# Autodesk Inventor assembly: Projekat
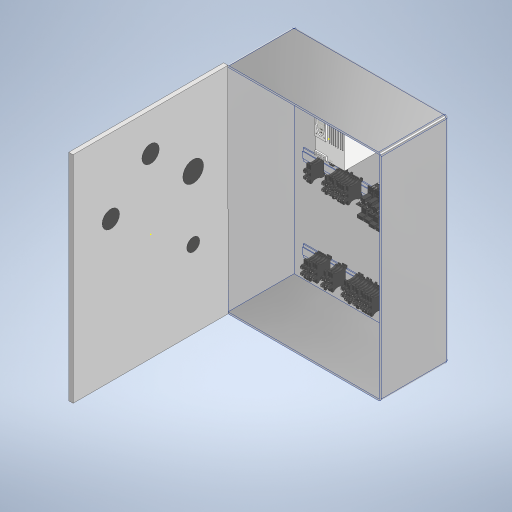
[picture p0: Inventor's stored thumbnail of the model, 512x512]
Saved by Autodesk Inventor 2023 (Build 270158000, 158)
## iProperties
Created: 2022-07-07
Part Number: Projekat
Document SubType Name: Assembly
Designer: User
Author: User
## Documents named in this file (9)
- C:\Users\User\Desktop\PMS\Seminarski rad\Inventor_sheme\Projekat.iam
- C:\Users\User\Desktop\PMS\Seminarski rad\Inventor_sheme\Ormar.ipt
- C:\Users\User\Desktop\PMS\Seminarski rad\Inventor_sheme\vrata.ipt
- C:\Users\User\Desktop\PMS\Seminarski rad\manja_sklopka\a9f89116.iam
- C:\Users\User\Desktop\PMS\Seminarski rad\Inventor_sheme\redna_stezaljka.ipt
- C:\Users\User\Desktop\PMS\Seminarski rad\sklopka\domf01204.iam
- C:\Users\User\Desktop\PMS\Seminarski rad\Inventor_sheme\napojna_jedinica_ABL8RPS24100.ipt
- C:\Users\User\Desktop\PMS\Seminarski rad\odvodnik_prenapona\a9a26500.iam
- C:\Users\User\Desktop\PMS\Seminarski rad\rsb_relay\rsb1a120f7pv.ipt
## Components (63 placed, 8 different names)
1. Ormar:1 — Mate:1, Mate:4, Mate:5, Mate:7, Mate:8, Mate:9, Mate:10, Mate:11, Mate:12, Mate:13, Mate:14, Mate:15, Mate:16, Mate:17, Mate:18, Mate:19, Mate:20, Mate:21, Mate:22, Mate:23, Mate:24, Mate:25, Mate:26, Mate:27, Mate:28, Mate:29, Mate:30, Mate:31, Mate:32, Mate:33, Mate:34, Mate:35, Mate:36, Mate:37, Mate:38, Mate:39, Mate:40, Mate:41, Mate:42, Mate:43, Mate:44, Mate:45, Mate:46, Mate:47, Mate:48, Mate:49, Mate:50, Mate:51, Mate:52, Mate:53, Mate:54, Mate:55, Mate:56, Mate:57, Mate:58, Mate:59, Mate:60, Mate:61, Mate:62, Mate:63, Mate:64, Mate:65, Mate:66
2. a9a26500:1 [sub-assembly] — Mate:8
3. domf01204:1 [sub-assembly] — Mate:5
4. a9f89116:1 [sub-assembly] — Mate:7
5. napojna_jedinica_ABL8RPS24100:1 — Mate:4
6. vrata:1 — Mate:1
7. redna_stezaljka:1 — Mate:9, Mate:11
8. redna_stezaljka:2 — Mate:10
9. redna_stezaljka:3 — Mate:12
10. redna_stezaljka:4 — Mate:13
11. redna_stezaljka:5 — Mate:15
12. redna_stezaljka:6 — Mate:16
13. redna_stezaljka:7 — Mate:14
14. redna_stezaljka:8 — Mate:24
15. redna_stezaljka:9 — Mate:23
16. redna_stezaljka:10 — Mate:21
17. redna_stezaljka:11 — Mate:22
18. redna_stezaljka:12 — Mate:17
19. redna_stezaljka:13 — Mate:20
20. redna_stezaljka:14 — Mate:18
21. redna_stezaljka:15 — Mate:19
22. rsb1a120f7pv:1 — Mate:25
23. rsb1a120f7pv:4 — Mate:26
24. rsb1a120f7pv:5 — Mate:27
25. rsb1a120f7pv:6 — Mate:28
26. rsb1a120f7pv:7 — Mate:29
27. rsb1a120f7pv:8 — Mate:30
28. redna_stezaljka:16 — Mate:39
29. redna_stezaljka:17 — Mate:36
30. redna_stezaljka:18 — Mate:35
31. redna_stezaljka:19 — Mate:38
32. redna_stezaljka:20 — Mate:40
33. redna_stezaljka:21 — Mate:41
34. redna_stezaljka:22 — Mate:37
35. redna_stezaljka:23 — Mate:34
36. redna_stezaljka:24 — Mate:33
37. redna_stezaljka:25 — Mate:31
38. redna_stezaljka:26 — Mate:32
39. redna_stezaljka:27 — Mate:47
40. redna_stezaljka:28 — Mate:48
41. redna_stezaljka:29 — Mate:46
42. redna_stezaljka:30 — Mate:49
43. redna_stezaljka:31 — Mate:45
44. redna_stezaljka:32 — Mate:44
45. redna_stezaljka:33 — Mate:43
46. redna_stezaljka:34 — Mate:42
47. redna_stezaljka:35 — Mate:66
48. redna_stezaljka:36 — Mate:64
49. redna_stezaljka:37 — Mate:60
50. redna_stezaljka:38 — Mate:63
51. redna_stezaljka:39 — Mate:59
52. redna_stezaljka:40 — Mate:57
53. redna_stezaljka:41 — Mate:58
54. redna_stezaljka:42 — Mate:65
55. redna_stezaljka:43 — Mate:62
56. redna_stezaljka:44 — Mate:56
57. redna_stezaljka:45 — Mate:61
58. redna_stezaljka:46 — Mate:55
59. redna_stezaljka:47 — Mate:54
60. redna_stezaljka:48 — Mate:53
61. redna_stezaljka:49 — Mate:51
62. redna_stezaljka:50 — Mate:52
63. redna_stezaljka:51 — Mate:50
## Relationships (63: Mate 63)
- Mate:1: Ormar:1 ↔ vrata:1
- Mate:4: Ormar:1 ↔ napojna_jedinica_ABL8RPS24100:1
- Mate:5: Ormar:1 ↔ domf01204:1
- Mate:7: Ormar:1 ↔ a9f89116:1
- Mate:8: Ormar:1 ↔ a9a26500:1
- Mate:9: Ormar:1 ↔ redna_stezaljka:1
- Mate:10: Ormar:1 ↔ redna_stezaljka:2
- Mate:11: Ormar:1 ↔ redna_stezaljka:1
- Mate:12: Ormar:1 ↔ redna_stezaljka:3
- Mate:13: Ormar:1 ↔ redna_stezaljka:4
- Mate:14: Ormar:1 ↔ redna_stezaljka:7
- Mate:15: Ormar:1 ↔ redna_stezaljka:5
- Mate:16: Ormar:1 ↔ redna_stezaljka:6
- Mate:17: Ormar:1 ↔ redna_stezaljka:12
- Mate:18: Ormar:1 ↔ redna_stezaljka:14
- Mate:19: Ormar:1 ↔ redna_stezaljka:15
- Mate:20: Ormar:1 ↔ redna_stezaljka:13
- Mate:21: Ormar:1 ↔ redna_stezaljka:10
- Mate:22: Ormar:1 ↔ redna_stezaljka:11
- Mate:23: Ormar:1 ↔ redna_stezaljka:9
- Mate:24: Ormar:1 ↔ redna_stezaljka:8
- Mate:25: Ormar:1 ↔ rsb1a120f7pv:1
- Mate:26: Ormar:1 ↔ rsb1a120f7pv:4
- Mate:27: Ormar:1 ↔ rsb1a120f7pv:5
- Mate:28: Ormar:1 ↔ rsb1a120f7pv:6
- Mate:29: Ormar:1 ↔ rsb1a120f7pv:7
- Mate:30: Ormar:1 ↔ rsb1a120f7pv:8
- Mate:31: Ormar:1 ↔ redna_stezaljka:25
- Mate:32: Ormar:1 ↔ redna_stezaljka:26
- Mate:33: Ormar:1 ↔ redna_stezaljka:24
- Mate:34: Ormar:1 ↔ redna_stezaljka:23
- Mate:35: Ormar:1 ↔ redna_stezaljka:18
- Mate:36: Ormar:1 ↔ redna_stezaljka:17
- Mate:37: Ormar:1 ↔ redna_stezaljka:22
- Mate:38: Ormar:1 ↔ redna_stezaljka:19
- Mate:39: Ormar:1 ↔ redna_stezaljka:16
- Mate:40: Ormar:1 ↔ redna_stezaljka:20
- Mate:41: Ormar:1 ↔ redna_stezaljka:21
- Mate:42: Ormar:1 ↔ redna_stezaljka:34
- Mate:43: Ormar:1 ↔ redna_stezaljka:33
- Mate:44: Ormar:1 ↔ redna_stezaljka:32
- Mate:45: Ormar:1 ↔ redna_stezaljka:31
- Mate:46: Ormar:1 ↔ redna_stezaljka:29
- Mate:47: Ormar:1 ↔ redna_stezaljka:27
- Mate:48: Ormar:1 ↔ redna_stezaljka:28
- Mate:49: Ormar:1 ↔ redna_stezaljka:30
- Mate:50: Ormar:1 ↔ redna_stezaljka:51
- Mate:51: Ormar:1 ↔ redna_stezaljka:49
- Mate:52: Ormar:1 ↔ redna_stezaljka:50
- Mate:53: Ormar:1 ↔ redna_stezaljka:48
- Mate:54: Ormar:1 ↔ redna_stezaljka:47
- Mate:55: Ormar:1 ↔ redna_stezaljka:46
- Mate:56: Ormar:1 ↔ redna_stezaljka:44
- Mate:57: Ormar:1 ↔ redna_stezaljka:40
- Mate:58: Ormar:1 ↔ redna_stezaljka:41
- Mate:59: Ormar:1 ↔ redna_stezaljka:39
- Mate:60: Ormar:1 ↔ redna_stezaljka:37
- Mate:61: Ormar:1 ↔ redna_stezaljka:45
- Mate:62: Ormar:1 ↔ redna_stezaljka:43
- Mate:63: Ormar:1 ↔ redna_stezaljka:38
- Mate:64: Ormar:1 ↔ redna_stezaljka:36
- Mate:65: Ormar:1 ↔ redna_stezaljka:42
- Mate:66: Ormar:1 ↔ redna_stezaljka:35
